# Autodesk Inventor assembly: UpperArm_MIR
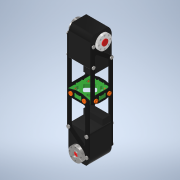
[picture p0: Inventor's stored thumbnail of the model, 180x180]
Saved by Autodesk Inventor 2020.4 (Build 244396000, 396)
## iProperties
Created: 2021-09-11
Part Number: UpperArm_MIR
Document SubType Name: Assembly
Designer: Masato Kubotera
Mass: 132.402 g
Surface Area: 432.665 cm^2
Volume: 110.152 cm^3
Density: 1.20199 g/cm^3
Author: Masato
## Documents named in this file (12)
- C:\Users\Masato\Documents\Inventor\CIT Brains_Inventor\OpenPlatform_ver3_0\UpperBody\Arm\UpperArm_MIR.iam
- C:\Users\Masato\Documents\Inventor\CIT Brains_Inventor\OpenPlatform_ver3_0\UpperBody\Arm\UpperArm_diagonal.ipt
- C:\Users\Masato\Documents\Inventor\CIT Brains_Inventor\OpenPlatform_ver3_0\ReadyMade\KONDO\B3M-SC-1040-A.ipt
- C:\Users\Masato\Documents\Inventor\CIT Brains_Inventor\OpenPlatform_ver3_0\ReadyMade\KONDO\ClampHorn.ipt
- C:\Users\Masato\Documents\Inventor\CIT Brains_Inventor\OpenPlatform_ver3_0\ReadyMade\KONDO\FreeHorn.ipt
- C:\Users\Masato\Documents\Inventor\CIT Brains_Inventor\OpenPlatform_ver3_0\ReadyMade\Screw\620103008.ipt
- C:\Users\Masato\Documents\Inventor\CIT Brains_Inventor\OpenPlatform_ver3_0\ReadyMade\KONDO\FreeHorn_Screw.ipt
- C:\Users\Masato\Documents\Inventor\CIT Brains_Inventor\OpenPlatform_ver3_0\UpperBody\Arm\UpperArm_side_frame.ipt
- C:\Users\Masato\Documents\Inventor\CIT Brains_Inventor\OpenPlatform_ver3_0\ReadyMade\Screw\M3-6.ipt
- C:\Users\Masato\Documents\Inventor\CIT Brains_Inventor\OpenPlatform_ver3_0\ReadyMade\Screw\M2_6-15.ipt
- C:\Users\Masato\Documents\Inventor\CIT Brains_Inventor\OpenPlatform_ver3_0\ReadyMade\Screw\M2_6-20.ipt
- C:\Users\Masato\Documents\Inventor\CIT Brains_Inventor\OpenPlatform_ver3_0\ReadyMade\InsertNut\IRU-304SW.ipt
## Components (43 placed, 11 different names)
1. B3M-SC-1040-A:1 — 挿入:45, 挿入:19, 挿入:18, 挿入:17, 挿入:22, 挿入:21, 挿入:20, 挿入:47, 挿入:41, 挿入:43, 角度:1
2. ClampHorn:1 — メイト:1, 挿入:41, 角度:1
3. FreeHorn:1 — 挿入:45, メイト:1
4. B3M-SC-1040-A:2 — 挿入:46, 挿入:25, 挿入:24, 挿入:23, 挿入:28, 挿入:27, 挿入:26, 挿入:48, 挿入:42, 挿入:44, 角度:2
5. ClampHorn:2 — メイト:2, 角度:2, 挿入:42
6. FreeHorn:2 — 挿入:46, メイト:2
7. UpperArm_diagonal:1 — フラッシュ:2, フラッシュ:1, メイト:3, 挿入:7, 挿入:8, 挿入:5, 挿入:6, 挿入:2, 挿入:1, 挿入:4, 挿入:3, 挿入:49, 挿入:50, 挿入:51, 挿入:52, 挿入:53, 挿入:54, 挿入:55, 挿入:56
8. UpperArm_side_frame:1 — 挿入:34, 挿入:33, 挿入:32, 挿入:25, 挿入:24, 挿入:23, 挿入:10, 挿入:9, 挿入:2, 挿入:1
9. UpperArm_side_frame:2 — 挿入:40, 挿入:39, 挿入:38, 挿入:28, 挿入:27, 挿入:26, 挿入:4, 挿入:3, 挿入:12, 挿入:11
10. UpperArm_side_frame:3 — 挿入:37, 挿入:36, 挿入:35, 挿入:19, 挿入:18, 挿入:17, 挿入:13, 挿入:14, 挿入:7, 挿入:8
11. UpperArm_side_frame:4 — 挿入:31, 挿入:30, 挿入:29, 挿入:22, 挿入:21, 挿入:20, 挿入:16, 挿入:15, 挿入:5, 挿入:6
12. 620103008:1 — 挿入:43
13. 620103008:2 — 挿入:44
14. FreeHorn_Screw:1 — 挿入:47
15. FreeHorn_Screw:2 — 挿入:48
16. M3-6:1 — 挿入:9
17. M3-6:2 — 挿入:10
18. M3-6:3 — 挿入:11
19. M3-6:4 — 挿入:12
20. M3-6:5 — 挿入:13
21. M3-6:6 — 挿入:14
22. M3-6:7 — 挿入:15
23. M3-6:8 — 挿入:16
24. M2_6-15:1 — 挿入:29
25. M2_6-15:2 — 挿入:30
26. M2_6-15:3 — 挿入:31
27. M2_6-15:4 — 挿入:32
28. M2_6-15:5 — 挿入:33
29. M2_6-15:6 — 挿入:34
30. M2_6-20:1 — 挿入:35
31. M2_6-20:2 — 挿入:36
32. M2_6-20:3 — 挿入:37
33. M2_6-20:4 — 挿入:39
34. M2_6-20:5 — 挿入:38
35. M2_6-20:6 — 挿入:40
36. IRU-304SW:8 — 挿入:56
37. IRU-304SW:7 — 挿入:55
38. IRU-304SW:6 — 挿入:54
39. IRU-304SW:5 — 挿入:53
40. IRU-304SW:4 — 挿入:52
41. IRU-304SW:3 — 挿入:51
42. IRU-304SW:2 — 挿入:50
43. IRU-304SW:1 — 挿入:49
## Relationships (63: Insert 56, Mate 4, Angle 2, Flush 1)
- フラッシュ:2 [Mate]: UpperArm_diagonal:1
- フラッシュ:1 [Flush]: UpperArm_diagonal:1
- メイト:3 [Mate]: UpperArm_diagonal:1
- 挿入:45 [Insert]: B3M-SC-1040-A:1 ↔ FreeHorn:1
- 挿入:46 [Insert]: B3M-SC-1040-A:2 ↔ FreeHorn:2
- 挿入:37 [Insert]: UpperArm_side_frame:3 ↔ M2_6-20:3
- 挿入:36 [Insert]: UpperArm_side_frame:3 ↔ M2_6-20:2
- 挿入:35 [Insert]: UpperArm_side_frame:3 ↔ M2_6-20:1
- 挿入:19 [Insert]: B3M-SC-1040-A:1 ↔ UpperArm_side_frame:3
- 挿入:18 [Insert]: B3M-SC-1040-A:1 ↔ UpperArm_side_frame:3
- 挿入:17 [Insert]: B3M-SC-1040-A:1 ↔ UpperArm_side_frame:3
- 挿入:13 [Insert]: UpperArm_side_frame:3 ↔ M3-6:5
- 挿入:14 [Insert]: UpperArm_side_frame:3 ↔ M3-6:6
- 挿入:7 [Insert]: UpperArm_diagonal:1 ↔ UpperArm_side_frame:3
- 挿入:8 [Insert]: UpperArm_diagonal:1 ↔ UpperArm_side_frame:3
- 挿入:31 [Insert]: UpperArm_side_frame:4 ↔ M2_6-15:3
- 挿入:30 [Insert]: UpperArm_side_frame:4 ↔ M2_6-15:2
- 挿入:29 [Insert]: UpperArm_side_frame:4 ↔ M2_6-15:1
- 挿入:22 [Insert]: B3M-SC-1040-A:1 ↔ UpperArm_side_frame:4
- 挿入:21 [Insert]: B3M-SC-1040-A:1 ↔ UpperArm_side_frame:4
- 挿入:20 [Insert]: B3M-SC-1040-A:1 ↔ UpperArm_side_frame:4
- 挿入:16 [Insert]: UpperArm_side_frame:4 ↔ M3-6:8
- 挿入:15 [Insert]: UpperArm_side_frame:4 ↔ M3-6:7
- 挿入:5 [Insert]: UpperArm_diagonal:1 ↔ UpperArm_side_frame:4
- 挿入:6 [Insert]: UpperArm_diagonal:1 ↔ UpperArm_side_frame:4
- 挿入:34 [Insert]: UpperArm_side_frame:1 ↔ M2_6-15:6
- 挿入:33 [Insert]: UpperArm_side_frame:1 ↔ M2_6-15:5
- 挿入:32 [Insert]: UpperArm_side_frame:1 ↔ M2_6-15:4
- 挿入:25 [Insert]: B3M-SC-1040-A:2 ↔ UpperArm_side_frame:1
- 挿入:24 [Insert]: B3M-SC-1040-A:2 ↔ UpperArm_side_frame:1
- 挿入:23 [Insert]: B3M-SC-1040-A:2 ↔ UpperArm_side_frame:1
- 挿入:10 [Insert]: UpperArm_side_frame:1 ↔ M3-6:2
- 挿入:9 [Insert]: UpperArm_side_frame:1 ↔ M3-6:1
- 挿入:2 [Insert]: UpperArm_diagonal:1 ↔ UpperArm_side_frame:1
- 挿入:1 [Insert]: UpperArm_diagonal:1 ↔ UpperArm_side_frame:1
- 挿入:40 [Insert]: UpperArm_side_frame:2 ↔ M2_6-20:6
- 挿入:39 [Insert]: UpperArm_side_frame:2 ↔ M2_6-20:4
- 挿入:38 [Insert]: UpperArm_side_frame:2 ↔ M2_6-20:5
- 挿入:28 [Insert]: B3M-SC-1040-A:2 ↔ UpperArm_side_frame:2
- 挿入:27 [Insert]: B3M-SC-1040-A:2 ↔ UpperArm_side_frame:2
- 挿入:26 [Insert]: B3M-SC-1040-A:2 ↔ UpperArm_side_frame:2
- 挿入:4 [Insert]: UpperArm_diagonal:1 ↔ UpperArm_side_frame:2
- 挿入:3 [Insert]: UpperArm_diagonal:1 ↔ UpperArm_side_frame:2
- 挿入:12 [Insert]: UpperArm_side_frame:2 ↔ M3-6:4
- 挿入:11 [Insert]: UpperArm_side_frame:2 ↔ M3-6:3
- 挿入:47 [Insert]: B3M-SC-1040-A:1 ↔ FreeHorn_Screw:1
- 挿入:48 [Insert]: B3M-SC-1040-A:2 ↔ FreeHorn_Screw:2
- メイト:1 [Mate]: ClampHorn:1 ↔ FreeHorn:1
- 挿入:41 [Insert]: B3M-SC-1040-A:1 ↔ ClampHorn:1
- メイト:2 [Mate]: ClampHorn:2 ↔ FreeHorn:2
- 挿入:42 [Insert]: B3M-SC-1040-A:2 ↔ ClampHorn:2
- 挿入:43 [Insert]: B3M-SC-1040-A:1 ↔ 620103008:1
- 挿入:44 [Insert]: B3M-SC-1040-A:2 ↔ 620103008:2
- 角度:1 [Angle] (0 deg): B3M-SC-1040-A:1 ↔ ClampHorn:1
- 角度:2 [Angle] (0 deg): B3M-SC-1040-A:2 ↔ ClampHorn:2
- 挿入:49 [Insert]: UpperArm_diagonal:1 ↔ IRU-304SW:1
- 挿入:50 [Insert]: UpperArm_diagonal:1 ↔ IRU-304SW:2
- 挿入:51 [Insert]: UpperArm_diagonal:1 ↔ IRU-304SW:3
- 挿入:52 [Insert]: UpperArm_diagonal:1 ↔ IRU-304SW:4
- 挿入:53 [Insert]: UpperArm_diagonal:1 ↔ IRU-304SW:5
- 挿入:54 [Insert]: UpperArm_diagonal:1 ↔ IRU-304SW:6
- 挿入:55 [Insert]: UpperArm_diagonal:1 ↔ IRU-304SW:7
- 挿入:56 [Insert]: UpperArm_diagonal:1 ↔ IRU-304SW:8
